# Autodesk Inventor assembly: bas frame
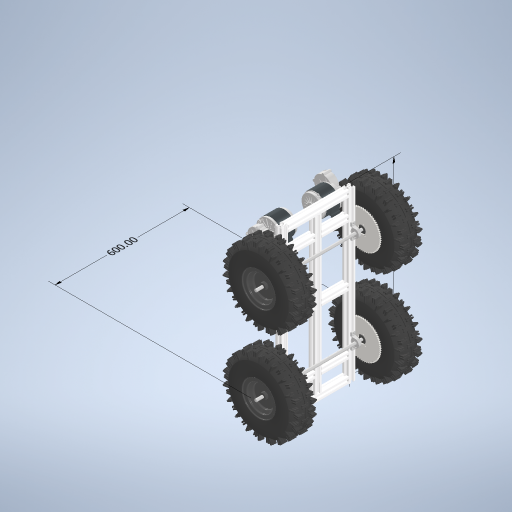
[picture p0: Inventor's stored thumbnail of the model, 512x512]
Saved by Autodesk Inventor 2023 (Build 270158000, 158)
## iProperties
Created: 2023-09-03
Part Number: bas frame
Document SubType Name: Assembly
Designer: sigit
Author: sigit
## Documents named in this file (9)
- D:\Kuliah\SEMESTER 7\Robot Semprot\Design\REVISI2\Assembly\bas frame.iam
- D:\Kuliah\SEMESTER 7\Robot Semprot\Design\REVISI2\Part\tslot 3030 750mm.ipt
- D:\Kuliah\SEMESTER 7\Robot Semprot\Design\REVISI2\Part\tslot 3030 270mm.ipt
- D:\Kuliah\SEMESTER 7\Robot Semprot\Design\REVISI2\Part\tslot 3030 690mm.ipt
- D:\Kuliah\SEMESTER 7\Robot Semprot\Design\REVISI2\Part\pillow block 12mm.ipt
- D:\Kuliah\SEMESTER 7\Robot Semprot\Design\REVISI2\Part\poros.ipt
- D:\Kuliah\SEMESTER 7\Robot Semprot\Design\REVISI2\Assembly\roda.iam
- D:\Kuliah\SEMESTER 7\Robot Semprot\Design\REVISI2\Assembly\Motor DC - MY1016Z.iam
- D:\Kuliah\SEMESTER 7\Robot Semprot\Design\REVISI2\Part\tslot 3030 120mm.ipt
## Components (23 placed, 8 different names)
1. tslot 3030 750mm:1 — Rotational:1, Rotational:3, Rotational:4, Rotational:11, Rigid:3, Rotational:16
2. tslot 3030 750mm:2 — Rotational:2, Rotational:5, Rotational:12, Rotational:13, Rotational:17
3. tslot 3030 270mm:1 — Rotational:1, Rotational:2, Rotational:14, Rotational:15
4. tslot 3030 270mm:2 — Rotational:3, Rigid:1
5. tslot 3030 690mm:1 — Rigid:1
6. poros:2 — Rotational:6, Rotational:19, Rotational:21
7. poros:3 — Rotational:7, Rotational:18, Rotational:20
8. tslot 3030 120mm:1 — Rotational:12
9. tslot 3030 120mm:2 — Rotational:11
10. tslot 3030 120mm:3 — Rotational:13
11. tslot 3030 120mm:4 — Rigid:3
12. Motor DC - MY1016Z:2 [sub-assembly] — Rotational:14
13. Motor DC - MY1016Z:3 [sub-assembly] — Rotational:15
14. tslot 3030 120mm:5 — Rotational:17
15. tslot 3030 120mm:6 — Rotational:16
16. roda:4 [sub-assembly] — Rotational:18
17. roda:5 [sub-assembly] — Rotational:19
18. roda:6 [sub-assembly] — Rotational:21
19. roda:7 [sub-assembly] — Rotational:20
20. pillow block 12mm:1 — Rotational:4
21. pillow block 12mm:2
22. pillow block 12mm:3 — Rotational:5, Rotational:6
23. pillow block 12mm:4 — Rotational:7
## Component patterns: (2 elements, first: pillow block 12mm:1), (2 elements, first: pillow block 12mm:3)
## Relationships (20: RevoluteJoint 18, WeldJoint 2)
- Rotational:1 [RevoluteJoint] (-9.486 mm): tslot 3030 750mm:1 ↔ tslot 3030 270mm:1
- Rotational:2 [RevoluteJoint] (9.486 mm): tslot 3030 750mm:2 ↔ tslot 3030 270mm:1
- Rotational:3 [RevoluteJoint] (-9.486 mm): tslot 3030 750mm:1 ↔ tslot 3030 270mm:2
- Rigid:1 [WeldJoint] (-9.486 mm): tslot 3030 270mm:2 ↔ tslot 3030 690mm:1
- Rotational:4 [RevoluteJoint] (9.486 mm): tslot 3030 750mm:1 ↔ pillow block 12mm:1
- Rotational:5 [RevoluteJoint] (9.486 mm): tslot 3030 750mm:2 ↔ pillow block 12mm:3
- Rotational:6 [RevoluteJoint] (460.5 mm): poros:2 ↔ pillow block 12mm:3
- Rotational:7 [RevoluteJoint] (460.5 mm): poros:3 ↔ pillow block 12mm:4
- Rotational:11 [RevoluteJoint] (-9.486 mm): tslot 3030 750mm:1 ↔ tslot 3030 120mm:2
- Rotational:12 [RevoluteJoint] (-9.486 mm): tslot 3030 750mm:2 ↔ tslot 3030 120mm:1
- Rotational:13 [RevoluteJoint] (-9.486 mm): tslot 3030 750mm:2 ↔ tslot 3030 120mm:3
- Rigid:3 [WeldJoint] (9.486 mm): tslot 3030 750mm:1 ↔ tslot 3030 120mm:4
- Rotational:14 [RevoluteJoint] (9.486 mm): tslot 3030 270mm:1 ↔ Motor DC - MY1016Z:2
- Rotational:15 [RevoluteJoint] (9.486 mm): tslot 3030 270mm:1 ↔ Motor DC - MY1016Z:3
- Rotational:16 [RevoluteJoint] (-9.486 mm): tslot 3030 750mm:1 ↔ tslot 3030 120mm:6
- Rotational:17 [RevoluteJoint] (-9.486 mm): tslot 3030 750mm:2 ↔ tslot 3030 120mm:5
- Rotational:18 [RevoluteJoint] (-123.25 mm): poros:3 ↔ roda:4
- Rotational:19 [RevoluteJoint] (-123.25 mm): poros:2 ↔ roda:5
- Rotational:20 [RevoluteJoint] (-123.25 mm): poros:3 ↔ roda:7
- Rotational:21 [RevoluteJoint] (-123.25 mm): poros:2 ↔ roda:6
